# Autodesk Inventor assembly: Assembly1
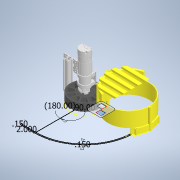
[picture p0: Inventor's stored thumbnail of the model, 180x180]
Saved by Autodesk Inventor 2020 (Build 240168000, 168)
## iProperties
Created: 2021-04-22
Part Number: Assembly1
Document SubType Name: Assembly
Designer: tdmp4
Author: tdmp4
## Documents named in this file (5)
- C:\Users\tdmp4\OneDrive\Documents\GitHub\CAD-2021-Ultimate_Goal\Shooter\Assembly1.iam
- C:\Users\tdmp4\OneDrive\Documents\GitHub\CAD-2021-Ultimate_Goal\Shooter\NewShooterBoard.ipt
- C:\Users\tdmp4\OneDrive\Documents\GitHub\CAD-2021-Ultimate_Goal\Shooter\NewShooterCup.ipt
- C:\Users\tdmp4\OneDrive\Documents\GitHub\CAD-2021-Ultimate_Goal\Shooter\RoofNewShooterCup.ipt
- C:\Users\tdmp4\OneDrive\Documents\GitHub\CAD-2021-Ultimate_Goal\Shooter\ShooterWheelSub.iam
## Components (4 placed, 4 different names)
1. NewShooterBoard:1 — Mate:1, Mate:2, Mate:3, Mate:8
2. NewShooterCup:1 — Mate:1, Mate:2, Mate:3, Mate:4, Mate:5, Mate:6, Mate:7
3. RoofNewShooterCup:1 — Mate:4, Mate:5, Mate:6, Mate:7
4. ShooterWheelSub:1 [sub-assembly] — Mate:8
## Relationships (8: Mate 8)
- Mate:1: NewShooterBoard:1 ↔ NewShooterCup:1
- Mate:2: NewShooterBoard:1 ↔ NewShooterCup:1
- Mate:3 (2.54 mm): NewShooterBoard:1 ↔ NewShooterCup:1
- Mate:4: NewShooterCup:1 ↔ RoofNewShooterCup:1
- Mate:5: NewShooterCup:1 ↔ RoofNewShooterCup:1
- Mate:6: NewShooterCup:1 ↔ RoofNewShooterCup:1
- Mate:7: NewShooterCup:1 ↔ RoofNewShooterCup:1
- Mate:8: NewShooterBoard:1 ↔ ShooterWheelSub:1
